# Autodesk Inventor assembly: arm j2 assemny
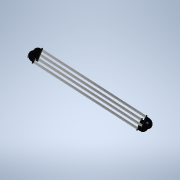
[picture p0: Inventor's stored thumbnail of the model, 180x180]
Saved by Autodesk Inventor 2020 (Build 240168000, 168)
## iProperties
Created: 2020-07-11
Part Number: arm j2 assemny
Document SubType Name: Assembly
Designer: Vikki
Mass: 15286.2 g
Surface Area: 29837.4 cm^2
Volume: 5661.55 cm^3
Density: 2.7 g/cm^3
Author: Vikki
## Documents named in this file (3)
- E:\project inventor pro\flipkart grid models\articulated arm\arm j2 assemny.iam
- E:\project inventor pro\flipkart grid models\articulated arm\arm j2.ipt
- E:\project inventor pro\flipkart grid models\articulated arm\2040ext 2200m.ipt
## Components (2 placed, 2 different names)
1. arm j2:1 — Mate:2, Mate:3, Flush:1, Flush:2, Flush:3
2. 2040ext 2200m:1 — Mate:2, Mate:3, Flush:1, Flush:2, Flush:3
## Relationships (5: Flush 3, Mate 2)
- Mate:2: arm j2:1 ↔ 2040ext 2200m:1
- Mate:3 (50 mm): arm j2:1 ↔ 2040ext 2200m:1
- Flush:1: arm j2:1 ↔ 2040ext 2200m:1
- Flush:2: arm j2:1 ↔ 2040ext 2200m:1
- Flush:3: arm j2:1 ↔ 2040ext 2200m:1
